# Autodesk Inventor assembly: Manipulator_Sterowniki_Robotow_I_czlon_obrotowy
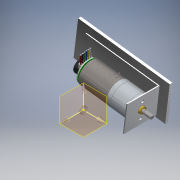
[picture p0: Inventor's stored thumbnail of the model, 180x180]
Saved by Autodesk Inventor 2019 (Build 230136000, 136)
## iProperties
Created: 2021-05-21
Part Number: Manipulator_Sterowniki_Robotow_I_czlon_obrotowy
Document SubType Name: Assembly
Designer: DOMEK
Sending System: SIEMENS PLM Software NX 1907
Preprocessor: ST-DEVELOPER v16.7
Title: Manipulator_Sterowniki_Robotów.stp
## Documents named in this file (4)
- D:\Manipulator\Inventor-20\Manipulator_Sterowniki_Robotow_I_czlon_obrotowy.iam
- D:\Manipulator\Inventor-20\Manipulator_DolnyHolderSilnika.ipt
- D:\Manipulator\Inventor-20\Manipulator_Handler_Silnikow.ipt
- D:\Manipulator\Inventor-20\25d-metal-gearmotor-172-227-encoder.ipt
## Components (3 placed, 3 different names)
1. Manipulator_DolnyHolderSilnika:1 — Flush:4
2. Manipulator_Handler_Silnikow:1 — Insert:4, Insert:5, Flush:4
3. 25d-metal-gearmotor-172-227-encoder:1 — Insert:4, Insert:5
## Relationships (3: Insert 2, Flush 1)
- Insert:4: Manipulator_Handler_Silnikow:1 ↔ 25d-metal-gearmotor-172-227-encoder:1
- Insert:5: Manipulator_Handler_Silnikow:1 ↔ 25d-metal-gearmotor-172-227-encoder:1
- Flush:4 (2 mm): Manipulator_DolnyHolderSilnika:1 ↔ Manipulator_Handler_Silnikow:1
